# Autodesk Inventor assembly: Selection
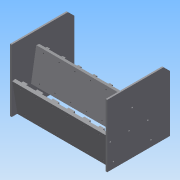
[picture p0: Inventor's stored thumbnail of the model, 180x180]
Saved by Autodesk Inventor 2018.1 (Build 221171000, 171)
## iProperties
Created: 2019-02-07
Part Number: Selection
Document SubType Name: Assembly
Designer: James
Author: James
## Documents named in this file (3)
- C:\Users\admin\Desktop\Ball Sorting Machine\CAD\Selection.iam
- C:\Users\admin\Desktop\Ball Sorting Machine\CAD\Selection_LHS.ipt
- C:\Users\admin\Desktop\Ball Sorting Machine\CAD\Selection_Ramp 1.iam
## Components (5 placed, 2 different names)
1. Selection_LHS:1 — Flush:1, Flush:2, Flush:3, Mate:2, Mate:3, Mate:4, Mate:5, Mate:6, Mate:7, Mate:8, Flush:9, Flush:10
2. Selection_Ramp 1:1 [sub-assembly] — Flush:7, Mate:2, Mate:3, Mate:9, Mate:10, Mate:11
3. Selection_Ramp 1:2 [sub-assembly] — Mate:4, Mate:5, Mate:6, Mate:12, Mate:13
4. Selection_Ramp 1:3 [sub-assembly] — Mate:7, Mate:8, Flush:8, Mate:14, Mate:15
5. Selection_LHS:2 — Mate:9, Flush:9, Flush:10, Mate:10, Mate:11, Mate:12, Mate:13, Mate:14, Mate:15
## Relationships (21: Mate 14, Flush 7)
- Flush:1: Selection_LHS:1
- Flush:2: Selection_LHS:1
- Flush:3: Selection_LHS:1
- Flush:7: Selection_Ramp 1:1
- Mate:2: Selection_LHS:1 ↔ Selection_Ramp 1:1
- Mate:3: Selection_LHS:1 ↔ Selection_Ramp 1:1
- Mate:4: Selection_LHS:1 ↔ Selection_Ramp 1:2
- Mate:5: Selection_LHS:1 ↔ Selection_Ramp 1:2
- Mate:6: Selection_LHS:1 ↔ Selection_Ramp 1:2
- Mate:7: Selection_LHS:1 ↔ Selection_Ramp 1:3
- Mate:8: Selection_LHS:1 ↔ Selection_Ramp 1:3
- Flush:8: Selection_Ramp 1:3
- Mate:9: Selection_Ramp 1:1 ↔ Selection_LHS:2
- Flush:9: Selection_LHS:1 ↔ Selection_LHS:2
- Flush:10: Selection_LHS:1 ↔ Selection_LHS:2
- Mate:10: Selection_Ramp 1:1 ↔ Selection_LHS:2
- Mate:11: Selection_Ramp 1:1 ↔ Selection_LHS:2
- Mate:12: Selection_Ramp 1:2 ↔ Selection_LHS:2
- Mate:13: Selection_Ramp 1:2 ↔ Selection_LHS:2
- Mate:14: Selection_Ramp 1:3 ↔ Selection_LHS:2
- Mate:15: Selection_Ramp 1:3 ↔ Selection_LHS:2
